# Autodesk Inventor assembly: Motor Gearbox and Shaft
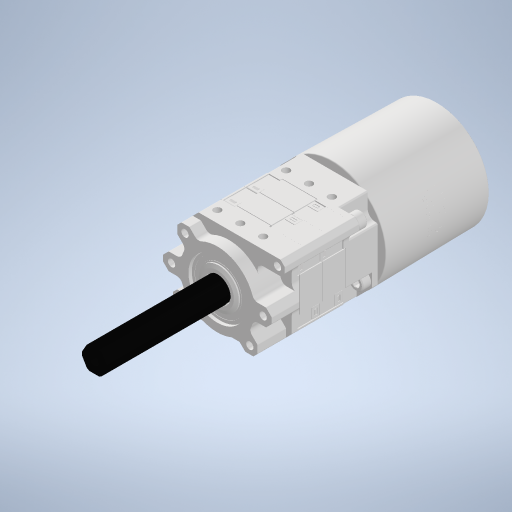
[picture p0: Inventor's stored thumbnail of the model, 512x512]
Saved by Autodesk Inventor 2023 (Build 270158000, 158)
## iProperties
Created: 2023-01-27
Part Number: Motor Gearbox and Shaft
Document SubType Name: Assembly
Designer: Gabriel - T3 CAD
Author: Gabriel - T3 CAD
## Documents named in this file (3)
- C:\Users\Gabriel - T3 CAD\Documents\GitHub\t3-CAD\T3-CAD\Current Season CAD\Swerve-DriveTrain-V2.1 (LongBot)\Winch assembly\Motor Gearbox and Shaft.iam
- C:\Users\Gabriel - T3 CAD\Documents\GitHub\t3-CAD\T3-CAD\Stock\Motors and Gearboxes\MAXPlanetary 2-Stage_Simplify_1.ipt
- C:\Users\Gabriel - T3 CAD\Documents\GitHub\t3-CAD\T3-CAD\Current Season CAD\Swerve-DriveTrain-V2.1 (LongBot)\Winch assembly\Winch shaft (Thunderhex).ipt
## Components (2 placed, 2 different names)
1. MAXPlanetary 2-Stage_Simplify_1:1 — Cylindrical:1, Rotational:1, Angle:1
2. Winch shaft (Thunderhex):1 — Cylindrical:1, Rotational:1, Angle:1
## Relationships (3: CylindricalJoint 1, RevoluteJoint 1, Angle 1)
- Cylindrical:1: MAXPlanetary 2-Stage_Simplify_1:1 ↔ Winch shaft (Thunderhex):1
- Rotational:1 [RevoluteJoint]: MAXPlanetary 2-Stage_Simplify_1:1 ↔ Winch shaft (Thunderhex):1
- Angle:1 (0 deg): MAXPlanetary 2-Stage_Simplify_1:1 ↔ Winch shaft (Thunderhex):1
